# Autodesk Inventor assembly: 74. Комплект первичного вала с кольцом после притирки
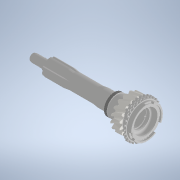
[picture p0: Inventor's stored thumbnail of the model, 180x180]
Saved by Autodesk Inventor 2021 (Build 250183000, 183)
## iProperties
Created: 2021-04-05
Part Number: 74. Комплект первичного вала с кольцом после притирки
Document SubType Name: Assembly
Designer: Данил
Author: Данил
## Documents named in this file (3)
- C:\Users\Данил\Desktop\Коробка передач\Детали\74. Комплект первичного вала с кольцом после притирки.iam
- C:\Users\Данил\Desktop\Коробка передач\Детали\64. Кольцо блокирующее.ipt
- C:\Users\Данил\Desktop\Коробка передач\Детали\68. Первичный вал.iam
## Components (2 placed, 2 different names)
1. 64. Кольцо блокирующее:1 — Совмещение:1, Совмещение:2
2. 68. Первичный вал:1 [sub-assembly] — Совмещение:1, Совмещение:2
## Relationships (2: Mate 2)
- Совмещение:1 [Mate]: 64. Кольцо блокирующее:1 ↔ 68. Первичный вал:1
- Совмещение:2 [Mate] (1.3 mm): 64. Кольцо блокирующее:1 ↔ 68. Первичный вал:1
